# Autodesk Inventor assembly: wheel with drive motor top_MIR
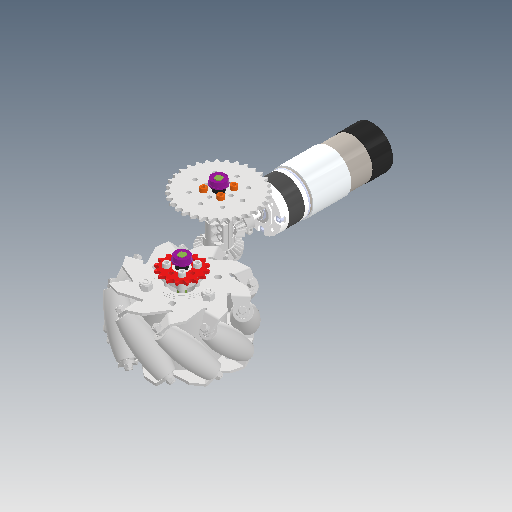
[picture p0: Inventor's stored thumbnail of the model, 512x512]
Saved by Autodesk Inventor 2020 (Build 240168000, 168)
## iProperties
Created: 2019-10-04
Part Number: wheel with drive motor top_MIR
Document SubType Name: Assembly
Designer: ball
Author: ball
## Documents named in this file (3)
- C:\FTC\FTC8863CAD\2019 Robot\Mecanum Drive Train\wheel with drive motor top_MIR.iam
- C:\FTC\FTC8863CAD\2019 Robot\Mecanum Drive Train\motor with bevil gear and sprocket_MIR.iam
- C:\FTC\FTC8863CAD\2019 Robot\Mecanum Drive Train\wheel with sprocket_MIR.iam
## Components (2 placed, 2 different names)
1. motor with bevil gear and sprocket_MIR:1 [sub-assembly] — Flush:3, Flush:4, Flush:2
2. wheel with sprocket_MIR:1 [sub-assembly] — Flush:3, Flush:4, Flush:2
## Relationships (3: Flush 3)
- Flush:3: motor with bevil gear and sprocket_MIR:1 ↔ wheel with sprocket_MIR:1
- Flush:4 (-76.2 mm): motor with bevil gear and sprocket_MIR:1 ↔ wheel with sprocket_MIR:1
- Flush:2 (-43.18 mm): motor with bevil gear and sprocket_MIR:1 ↔ wheel with sprocket_MIR:1
